# Autodesk Inventor assembly: part1
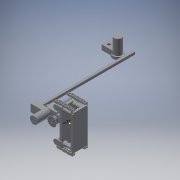
[picture p0: Inventor's stored thumbnail of the model, 180x180]
Saved by Autodesk Inventor 2019 (Build 230136000, 136)
## iProperties
Created: 2021-08-30
Part Number: part1
Material: 一般
Document SubType Name: Assembly
Designer: yuta
Author: yuta
## Documents named in this file (19)
- C:\Users\yuta\Documents\キャチロボ\part1.iam
- C:\Users\yuta\Documents\キャチロボ\Part10.ipt
- C:\Users\yuta\Documents\ACCURATE_C20623753d\ACCURATE_C206383d\C206 (38)3d.ipt
- C:\Users\yuta\Documents\キャチロボ\Part9.ipt
- C:\Users\yuta\Documents\キャチロボ\Part11.ipt
- C:\Users\yuta\Documents\AIS2019\06B - 1 RP- Pin 2.ipt
- C:\Users\yuta\Documents\AIS2019\Standard Chain06B1RP.iam
- C:\Users\yuta\Documents\キャチロボ\Part12.ipt
- C:\Users\yuta\Documents\キャチロボ\Part13.ipt
- C:\Users\yuta\Documents\キャチロボ\Part14.ipt
- C:\Users\yuta\Documents\AIS2019\06B - 1 RP - Body.ipt
- C:\Users\yuta\Documents\キャチロボ\Assembly3.iam
- C:\Users\yuta\Documents\キャチロボ\Part20.ipt
- C:\Users\yuta\Documents\キャチロボ\Part18.ipt
- C:\Users\yuta\Documents\キャチロボ\Part26.ipt
- C:\Users\yuta\Documents\キャチロボ\Part25.ipt
- C:\Users\yuta\Documents\キャチロボ\Assembly3,1.iam
- C:\Users\yuta\Documents\キャチロボ\Part27.ipt
- C:\Users\yuta\Documents\キャチロボ\Part28.ipt
## Components (41 placed, 18 different names)
1. Part10:1 — メイト:1, メイト:2, メイト:3, メイト:4, メイト:32, メイト:33, メイト:37, メイト:38, メイト:42, メイト:43, メイト:45, メイト:46, メイト:56
2. C206 (38)3d:1 — メイト:1, メイト:5
3. C206 (38)3d:2 — メイト:2
4. C206 (38)3d:3 — メイト:4
5. C206 (38)3d:4 — メイト:3
6. Part9:1 — メイト:5, メイト:6, フラッシュ:1, メイト:15, メイト:16, メイト:17, メイト:18, メイト:26, メイト:27
7. Part11:3 — メイト:6, フラッシュ:1, メイト:7, メイト:8
8. 06B - 1 RP- Pin 2:1 — メイト:7, メイト:8, メイト:9
9. Standard Chain06B1RP:1 [sub-assembly] — メイト:9
10. Part11:4 — メイト:17, メイト:18, メイト:19, メイト:20, メイト:24
11. Part11:5 — メイト:15, メイト:16, メイト:21, メイト:22, メイト:25
12. 06B - 1 RP- Pin 2:3 — メイト:19, メイト:20, メイト:23
13. 06B - 1 RP- Pin 2:4 — メイト:21, メイト:22
14. Standard Chain06B1RP:3 [sub-assembly] — メイト:25, メイト:53
15. Standard Chain06B1RP:4 [sub-assembly] — メイト:23, メイト:24, メイト:52
16. Part11:6 — メイト:26, メイト:27, メイト:28, メイト:29, メイト:31
17. 06B - 1 RP- Pin 2:5 — メイト:28, メイト:29, メイト:30
18. Standard Chain06B1RP:5 [sub-assembly] — メイト:30, メイト:31
19. Part12:1 — メイト:32, メイト:33, メイト:39, メイト:49
20. Part13:1 — メイト:39, メイト:40, メイト:48
21. Part13:2 — メイト:44, メイト:47, メイト:50
22. Part12:5 — メイト:37, メイト:38, メイト:40
23. Part12:6 — メイト:42, メイト:43, メイト:44
24. Part12:7 — メイト:45, メイト:46, メイト:47, メイト:51
25. Part14:1 — メイト:48, メイト:49
26. Part14:2 — メイト:50, メイト:51
27. 06B - 1 RP - Body:1 — メイト:52, メイト:54
28. 06B - 1 RP - Body:2 — メイト:53, メイト:55
29. 06B - 1 RP- Pin 2:6 — メイト:54
30. 06B - 1 RP- Pin 2:7 — メイト:55
31. Assembly3:1 [sub-assembly] — メイト:58
32. Part20:1 — メイト:56, メイト:57
33. Part18:1 — メイト:57, メイト:58, メイト:59, フラッシュ:2
34. Part26:1 — メイト:59, フラッシュ:2, メイト:60, フラッシュ:3
35. Part25:1 — メイト:60, フラッシュ:3, メイト:61, メイト:63
36. Assembly3,1:1 [sub-assembly] — メイト:61, メイト:62
37. Part27:1 — メイト:62, メイト:63, メイト:64, フラッシュ:4
38. Part28:1 — メイト:64, フラッシュ:4
39. Part25:2 — メイト:65
40. Assembly3,1:2 [sub-assembly] — メイト:65, メイト:66
41. Part27:3 — メイト:66
## Relationships (61: Mate 57, Flush 4)
- メイト:1 [Mate]: Part10:1 ↔ C206 (38)3d:1
- メイト:2 [Mate]: Part10:1 ↔ C206 (38)3d:2
- メイト:3 [Mate]: Part10:1 ↔ C206 (38)3d:4
- メイト:4 [Mate]: Part10:1 ↔ C206 (38)3d:3
- メイト:5 [Mate]: C206 (38)3d:1 ↔ Part9:1
- メイト:6 [Mate]: Part9:1 ↔ Part11:3
- フラッシュ:1 [Flush]: Part9:1 ↔ Part11:3
- メイト:7 [Mate]: Part11:3 ↔ 06B - 1 RP- Pin 2:1
- メイト:8 [Mate] (-1 mm): Part11:3 ↔ 06B - 1 RP- Pin 2:1
- メイト:9 [Mate]: 06B - 1 RP- Pin 2:1 ↔ Standard Chain06B1RP:1
- メイト:15 [Mate]: Part9:1 ↔ Part11:5
- メイト:16 [Mate]: Part9:1 ↔ Part11:5
- メイト:17 [Mate]: Part9:1 ↔ Part11:4
- メイト:18 [Mate]: Part9:1 ↔ Part11:4
- メイト:19 [Mate]: Part11:4 ↔ 06B - 1 RP- Pin 2:3
- メイト:20 [Mate] (1 mm): Part11:4 ↔ 06B - 1 RP- Pin 2:3
- メイト:21 [Mate]: Part11:5 ↔ 06B - 1 RP- Pin 2:4
- メイト:22 [Mate] (-1 mm): Part11:5 ↔ 06B - 1 RP- Pin 2:4
- メイト:23 [Mate]: 06B - 1 RP- Pin 2:3 ↔ Standard Chain06B1RP:4
- メイト:24 [Mate]: Part11:4 ↔ Standard Chain06B1RP:4
- メイト:25 [Mate]: Part11:5 ↔ Standard Chain06B1RP:3
- メイト:26 [Mate]: Part9:1 ↔ Part11:6
- メイト:27 [Mate]: Part9:1 ↔ Part11:6
- メイト:28 [Mate]: Part11:6 ↔ 06B - 1 RP- Pin 2:5
- メイト:29 [Mate] (1 mm): Part11:6 ↔ 06B - 1 RP- Pin 2:5
- メイト:30 [Mate]: 06B - 1 RP- Pin 2:5 ↔ Standard Chain06B1RP:5
- メイト:31 [Mate]: Part11:6 ↔ Standard Chain06B1RP:5
- メイト:32 [Mate]: Part10:1 ↔ Part12:1
- メイト:33 [Mate]: Part10:1 ↔ Part12:1
- メイト:37 [Mate]: Part10:1 ↔ Part12:5
- メイト:38 [Mate]: Part10:1 ↔ Part12:5
- メイト:39 [Mate]: Part12:1 ↔ Part13:1
- メイト:40 [Mate]: Part13:1 ↔ Part12:5
- メイト:42 [Mate]: Part10:1 ↔ Part12:6
- メイト:43 [Mate]: Part10:1 ↔ Part12:6
- メイト:44 [Mate]: Part13:2 ↔ Part12:6
- メイト:45 [Mate]: Part10:1 ↔ Part12:7
- メイト:46 [Mate]: Part10:1 ↔ Part12:7
- メイト:47 [Mate]: Part13:2 ↔ Part12:7
- メイト:48 [Mate]: Part13:1 ↔ Part14:1
- メイト:49 [Mate]: Part12:1 ↔ Part14:1
- メイト:50 [Mate]: Part13:2 ↔ Part14:2
- メイト:51 [Mate]: Part12:7 ↔ Part14:2
- メイト:52 [Mate]: Standard Chain06B1RP:4 ↔ 06B - 1 RP - Body:1
- メイト:53 [Mate]: Standard Chain06B1RP:3 ↔ 06B - 1 RP - Body:2
- メイト:54 [Mate]: 06B - 1 RP - Body:1 ↔ 06B - 1 RP- Pin 2:6
- メイト:55 [Mate]: 06B - 1 RP - Body:2 ↔ 06B - 1 RP- Pin 2:7
- メイト:56 [Mate]: Part10:1 ↔ Part20:1
- メイト:57 [Mate]: Part20:1 ↔ Part18:1
- メイト:58 [Mate]: Assembly3:1 ↔ Part18:1
- メイト:59 [Mate]: Part18:1 ↔ Part26:1
- フラッシュ:2 [Flush]: Part18:1 ↔ Part26:1
- メイト:60 [Mate]: Part26:1 ↔ Part25:1
- フラッシュ:3 [Flush] (5 mm): Part26:1 ↔ Part25:1
- メイト:61 [Mate]: Part25:1 ↔ Assembly3,1:1
- メイト:62 [Mate]: Assembly3,1:1 ↔ Part27:1
- メイト:63 [Mate]: Part25:1 ↔ Part27:1
- メイト:64 [Mate]: Part27:1 ↔ Part28:1
- フラッシュ:4 [Flush]: Part27:1 ↔ Part28:1
- メイト:65 [Mate]: Part25:2 ↔ Assembly3,1:2
- メイト:66 [Mate]: Assembly3,1:2 ↔ Part27:3
